# Autodesk Inventor assembly: asm
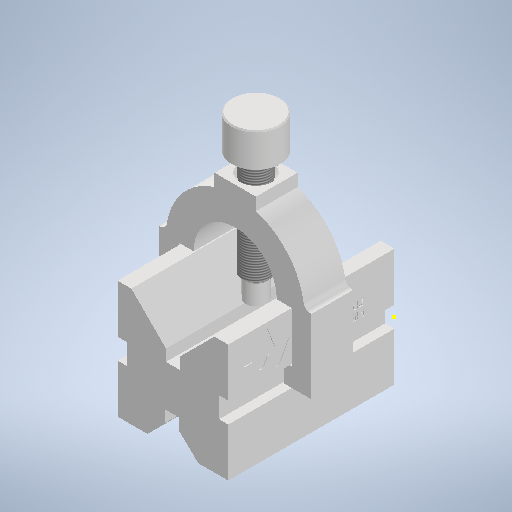
[picture p0: Inventor's stored thumbnail of the model, 512x512]
Saved by Autodesk Inventor 2025 (Build 290162000, 162)
## iProperties
Created: 2025-04-24
Part Number: asm
Document SubType Name: Assembly
Designer: jakub
Author: jakub
## Documents named in this file (4)
- C:\Users\jakub\Documents\Inventor\bitchsdd\asm.iam
- C:\Users\jakub\Documents\Inventor\bitchsdd\NECO.ipt
- C:\Users\jakub\Documents\Inventor\bitchsdd\picovina.ipt
- C:\Users\jakub\Documents\Inventor\bitchsdd\Sroub.ipt
## Components (3 placed, 3 different names)
1. NECO:1 — Slider:1, Rotational:1
2. picovina:1 — Slider:1
3. Sroub:1 — Rotational:1
## Relationships (2: TranslationJoint 1, RevoluteJoint 1)
- Slider:1 [TranslationJoint] (1 mm): NECO:1 ↔ picovina:1
- Rotational:1 [RevoluteJoint] (7.5 mm): NECO:1 ↔ Sroub:1
